# Autodesk Inventor assembly: fourbardraft
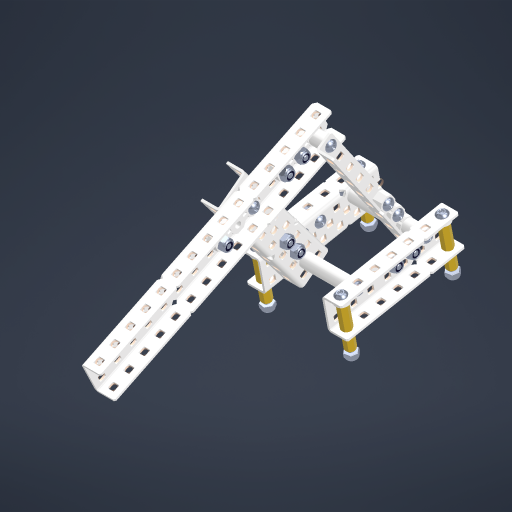
[picture p0: Inventor's stored thumbnail of the model, 512x512]
Saved by Autodesk Inventor 2023 (Build 270158000, 158)
## iProperties
Created: 2023-08-09
Part Number: fourbardraft
Document SubType Name: Assembly
Designer: srbel
Author: srbel
## Documents named in this file (20)
- C:\CAD\OverUnderCAD\Drive\fourbardraft.iam
- C:\CAD\OverUnderCAD\VEX-CAD-Inventor-1.4.0\Structure\C Channel\Aluminum 1x2x1\Alu C 1x2x1x6.ipt
- C:\CAD\OverUnderCAD\VEX-CAD-Inventor-1.4.0\Motion\Spacers\Spacer Nylon .313 OD\NSpacer .313 OD x .250.ipt
- C:\CAD\OverUnderCAD\VEX-CAD-Inventor-1.4.0\Motion\Spacers\Spacer Nylon .313 OD.ipt
- C:\CAD\OverUnderCAD\VEX-CAD-Inventor-1.4.0\Motion\Spacers\Spacer Nylon .313 OD\NSpacer .313 OD x .375.ipt
- C:\CAD\OverUnderCAD\VEX-CAD-Inventor-1.4.0\Motion\Spacers\Washer Teflon\TWasher .375 OD x .06250.ipt
- C:\CAD\OverUnderCAD\VEX-CAD-Inventor-1.4.0\Motion\Spacers\Washer Teflon.ipt
- C:\CAD\OverUnderCAD\VEX-CAD-Inventor-1.4.0\Structure\Hardware\Screw Steel - Star\SScrew Star Threaded .500.ipt
- C:\CAD\OverUnderCAD\VEX-CAD-Inventor-1.4.0\Structure\Hardware\Screw Steel - Star.ipt
- C:\CAD\OverUnderCAD\VEX-CAD-Inventor-1.4.0\Structure\Hardware\Screw Steel - Star\SScrew Star Threaded 2.500.ipt
- C:\CAD\OverUnderCAD\VEX-CAD-Inventor-1.4.0\Motion\Spacers\Spacer Nylon .313 OD\NSpacer .313 OD x .500.ipt
- C:\CAD\OverUnderCAD\VEX-CAD-Inventor-1.4.0\Structure\Hardware\Screw Steel - Star\SScrew Star Threaded .875.ipt
- C:\CAD\OverUnderCAD\Drive\fourbarintakebearing_MIR2_MIR1.iam
- C:\CAD\OverUnderCAD\Drive\fourbarintakebearing_MIR_MIR1_MIR1.iam
- C:\CAD\OverUnderCAD\VEX-CAD-Inventor-1.4.0\Motion\Shaft LS\Bearing Flat_MIR5_MIR1.ipt
- C:\CAD\OverUnderCAD\VEX-CAD-Inventor-1.4.0\Structure\C Channel\Aluminum 1x2x1\Alu C 1x2x1x8_MIR2_MIR1.ipt
- C:\CAD\OverUnderCAD\VEX-CAD-Inventor-1.4.0\Structure\Angle\Aluminum\1x1\Alu Angle 1x1x8_MIR2_MIR1.ipt
- C:\CAD\OverUnderCAD\VEX-CAD-Inventor-1.4.0\Structure\C Channel\Aluminum 1x2x1\Alu C 1x2x1x15_MIR1_MIR1.ipt
- C:\CAD\OverUnderCAD\VEX-CAD-Inventor-1.4.0\Motion\Shaft LS\Bearing Flat_MIR3_MIR1_MIR1.ipt
- C:\CAD\OverUnderCAD\VEX-CAD-Inventor-1.4.0\Structure\Hardware\Nut Thin Nylock_MIR7_MIR1_MIR1.ipt
## Components (48 placed, 16 different names)
1. Alu C 1x2x1x6:1
2. fourbarintakebearing_MIR2_MIR1:1 [sub-assembly] — Insert:173, Insert:199, Insert:201, Insert:202
3. fourbarintakebearing_MIR_MIR1_MIR1:1 [sub-assembly] — Insert:177, Insert:183, Insert:185, Insert:186, Insert:196, Insert:219
4. Bearing Flat_MIR5_MIR1:1 — Insert:170, Insert:171, Insert:172, Insert:192, Insert:193
5. Alu C 1x2x1x8_MIR2_MIR1:1 — Insert:170, Insert:171, Insert:178, Insert:194, Insert:195, Insert:217
6. NSpacer .313 OD x .250:33 — Insert:172, Insert:173
7. Bearing Flat_MIR5_MIR1:2 — Insert:174, Insert:175, Insert:176, Insert:189, Insert:190
8. Alu Angle 1x1x8_MIR2_MIR1:1 — Insert:174, Insert:175, Insert:182, Insert:188, Insert:191, Insert:203, Insert:206
9. NSpacer .313 OD x .250:34 — Insert:176, Insert:177
10. Alu C 1x2x1x15_MIR1_MIR1:1 — Insert:178, Insert:179, Insert:180, Insert:207, Insert:209, Insert:212, Insert:214, Insert:215, Insert:221
11. Bearing Flat_MIR5_MIR1:3 — Insert:179, Insert:180, Insert:181, Insert:208, Insert:210
12. NSpacer .313 OD x .375:35 — Insert:181, Insert:182
13. Bearing Flat_MIR3_MIR1_MIR1:1 — Insert:183, Insert:184, Insert:187, Insert:200
14. Nut Thin Nylock_MIR7_MIR1_MIR1:1 — Insert:184
15. SScrew Star Threaded .500:28 — Insert:185
16. SScrew Star Threaded .500:29 — Insert:186
17. Nut Thin Nylock_MIR7_MIR1_MIR1:2 — Insert:187
18. Nut Thin Nylock_MIR7_MIR1_MIR1:3 — Insert:188
19. SScrew Star Threaded .500:30 — Insert:189
20. SScrew Star Threaded .500:31 — Insert:190
21. Nut Thin Nylock_MIR7_MIR1_MIR1:4 — Insert:191
22. SScrew Star Threaded .500:32 — Insert:192
23. SScrew Star Threaded .500:33 — Insert:193
24. Nut Thin Nylock_MIR7_MIR1_MIR1:5 — Insert:194
25. Nut Thin Nylock_MIR7_MIR1_MIR1:6 — Insert:195
26. Nut Thin Nylock_MIR7_MIR1_MIR1:7 — Insert:197
27. TWasher .375 OD x .06250:9 — Insert:196, Insert:197
28. Nut Thin Nylock_MIR7_MIR1_MIR1:8 — Insert:198
29. TWasher .375 OD x .06250:10 — Insert:198, Insert:199
30. SScrew Star Threaded 2.500:34 — Insert:200
31. SScrew Star Threaded 2.500:35 — Insert:201
32. NSpacer .313 OD x .250:36 — Insert:202, Insert:205
33. NSpacer .313 OD x .500:37 — Insert:203, Insert:204
34. NSpacer .313 OD x .500:38 — Insert:204, Insert:205
35. SScrew Star Threaded .875:36 — Insert:206
36. SScrew Star Threaded .500:37 — Insert:207
37. Nut Thin Nylock_MIR7_MIR1_MIR1:9 — Insert:208
38. SScrew Star Threaded .500:38 — Insert:209
39. Nut Thin Nylock_MIR7_MIR1_MIR1:10 — Insert:210
40. SScrew Star Threaded .500:39 — Insert:211, Insert:216
41. Nut Thin Nylock_MIR7_MIR1_MIR1:11 — Insert:211
42. SScrew Star Threaded .500:40 — Insert:212, Insert:213
43. Nut Thin Nylock_MIR7_MIR1_MIR1:12 — Insert:213
44. Bearing Flat_MIR5_MIR1:4 — Insert:214, Insert:215, Insert:216
45. NSpacer .313 OD x .500:39 — Insert:217, Insert:218
46. NSpacer .313 OD x .250:40 — Insert:218, Insert:220
47. NSpacer .313 OD x .500:41 — Insert:219, Insert:220
48. Nut Thin Nylock_MIR7_MIR1_MIR1:13 — Insert:221
## Relationships (52: Insert 52)
- Insert:170: Bearing Flat_MIR5_MIR1:1 ↔ Alu C 1x2x1x8_MIR2_MIR1:1
- Insert:171: Bearing Flat_MIR5_MIR1:1 ↔ Alu C 1x2x1x8_MIR2_MIR1:1
- Insert:172: Bearing Flat_MIR5_MIR1:1 ↔ NSpacer .313 OD x .250:33
- Insert:173: fourbarintakebearing_MIR2_MIR1:1 ↔ NSpacer .313 OD x .250:33
- Insert:174: Bearing Flat_MIR5_MIR1:2 ↔ Alu Angle 1x1x8_MIR2_MIR1:1
- Insert:175: Bearing Flat_MIR5_MIR1:2 ↔ Alu Angle 1x1x8_MIR2_MIR1:1
- Insert:176: Bearing Flat_MIR5_MIR1:2 ↔ NSpacer .313 OD x .250:34
- Insert:177: fourbarintakebearing_MIR_MIR1_MIR1:1 ↔ NSpacer .313 OD x .250:34
- Insert:178: Alu C 1x2x1x8_MIR2_MIR1:1 ↔ Alu C 1x2x1x15_MIR1_MIR1:1
- Insert:179: Alu C 1x2x1x15_MIR1_MIR1:1 ↔ Bearing Flat_MIR5_MIR1:3
- Insert:180: Alu C 1x2x1x15_MIR1_MIR1:1 ↔ Bearing Flat_MIR5_MIR1:3
- Insert:181: Bearing Flat_MIR5_MIR1:3 ↔ NSpacer .313 OD x .375:35
- Insert:182: Alu Angle 1x1x8_MIR2_MIR1:1 ↔ NSpacer .313 OD x .375:35
- Insert:183: fourbarintakebearing_MIR_MIR1_MIR1:1 ↔ Bearing Flat_MIR3_MIR1_MIR1:1
- Insert:184: Bearing Flat_MIR3_MIR1_MIR1:1 ↔ Nut Thin Nylock_MIR7_MIR1_MIR1:1
- Insert:185: fourbarintakebearing_MIR_MIR1_MIR1:1 ↔ SScrew Star Threaded .500:28
- Insert:186: fourbarintakebearing_MIR_MIR1_MIR1:1 ↔ SScrew Star Threaded .500:29
- Insert:187: Bearing Flat_MIR3_MIR1_MIR1:1 ↔ Nut Thin Nylock_MIR7_MIR1_MIR1:2
- Insert:188: Alu Angle 1x1x8_MIR2_MIR1:1 ↔ Nut Thin Nylock_MIR7_MIR1_MIR1:3
- Insert:189: Bearing Flat_MIR5_MIR1:2 ↔ SScrew Star Threaded .500:30
- Insert:190: Bearing Flat_MIR5_MIR1:2 ↔ SScrew Star Threaded .500:31
- Insert:191: Alu Angle 1x1x8_MIR2_MIR1:1 ↔ Nut Thin Nylock_MIR7_MIR1_MIR1:4
- Insert:192: Bearing Flat_MIR5_MIR1:1 ↔ SScrew Star Threaded .500:32
- Insert:193: Bearing Flat_MIR5_MIR1:1 ↔ SScrew Star Threaded .500:33
- Insert:194: Alu C 1x2x1x8_MIR2_MIR1:1 ↔ Nut Thin Nylock_MIR7_MIR1_MIR1:5
- Insert:195: Alu C 1x2x1x8_MIR2_MIR1:1 ↔ Nut Thin Nylock_MIR7_MIR1_MIR1:6
- Insert:196: fourbarintakebearing_MIR_MIR1_MIR1:1 ↔ TWasher .375 OD x .06250:9
- Insert:197: Nut Thin Nylock_MIR7_MIR1_MIR1:7 ↔ TWasher .375 OD x .06250:9
- Insert:198: Nut Thin Nylock_MIR7_MIR1_MIR1:8 ↔ TWasher .375 OD x .06250:10
- Insert:199: fourbarintakebearing_MIR2_MIR1:1 ↔ TWasher .375 OD x .06250:10
- Insert:200: Bearing Flat_MIR3_MIR1_MIR1:1 ↔ SScrew Star Threaded 2.500:34
- Insert:201: fourbarintakebearing_MIR2_MIR1:1 ↔ SScrew Star Threaded 2.500:35
- Insert:202: fourbarintakebearing_MIR2_MIR1:1 ↔ NSpacer .313 OD x .250:36
- Insert:203: Alu Angle 1x1x8_MIR2_MIR1:1 ↔ NSpacer .313 OD x .500:37
- Insert:204: NSpacer .313 OD x .500:37 ↔ NSpacer .313 OD x .500:38
- Insert:205: NSpacer .313 OD x .250:36 ↔ NSpacer .313 OD x .500:38
- Insert:206: Alu Angle 1x1x8_MIR2_MIR1:1 ↔ SScrew Star Threaded .875:36
- Insert:207: Alu C 1x2x1x15_MIR1_MIR1:1 ↔ SScrew Star Threaded .500:37
- Insert:208: Bearing Flat_MIR5_MIR1:3 ↔ Nut Thin Nylock_MIR7_MIR1_MIR1:9
- Insert:209: Alu C 1x2x1x15_MIR1_MIR1:1 ↔ SScrew Star Threaded .500:38
- Insert:210: Bearing Flat_MIR5_MIR1:3 ↔ Nut Thin Nylock_MIR7_MIR1_MIR1:10
- Insert:211 (8.3185 mm): SScrew Star Threaded .500:39 ↔ Nut Thin Nylock_MIR7_MIR1_MIR1:11
- Insert:212: Alu C 1x2x1x15_MIR1_MIR1:1 ↔ SScrew Star Threaded .500:40
- Insert:213 (8.3185 mm): SScrew Star Threaded .500:40 ↔ Nut Thin Nylock_MIR7_MIR1_MIR1:12
- Insert:214: Alu C 1x2x1x15_MIR1_MIR1:1 ↔ Bearing Flat_MIR5_MIR1:4
- Insert:215: Alu C 1x2x1x15_MIR1_MIR1:1 ↔ Bearing Flat_MIR5_MIR1:4
- Insert:216: SScrew Star Threaded .500:39 ↔ Bearing Flat_MIR5_MIR1:4
- Insert:217: Alu C 1x2x1x8_MIR2_MIR1:1 ↔ NSpacer .313 OD x .500:39
- Insert:218: NSpacer .313 OD x .500:39 ↔ NSpacer .313 OD x .250:40
- Insert:219: fourbarintakebearing_MIR_MIR1_MIR1:1 ↔ NSpacer .313 OD x .500:41
- Insert:220: NSpacer .313 OD x .250:40 ↔ NSpacer .313 OD x .500:41
- Insert:221: Alu C 1x2x1x15_MIR1_MIR1:1 ↔ Nut Thin Nylock_MIR7_MIR1_MIR1:13
